# Autodesk Inventor assembly: ACTUADOR_LINEAL
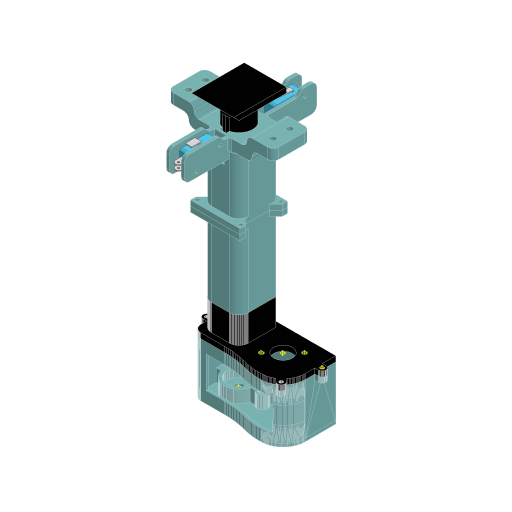
[picture p0: Inventor's stored thumbnail of the model, 512x512]
Saved by Autodesk Inventor 2024 (Build 280153000, 153)
## iProperties
Created: 2024-08-20
Part Number: ACTUADOR_LINEAL
Document SubType Name: Assembly
Designer: Jhuliams
Author: Jhuliams
## Documents named in this file (8)
- C:\Users\Jhuliams\Documents\GitHub\RECICLADOR_MODELO_3D\ACTUADOR_PARA_EMPUJAR_HACIA_ABAJO\ACTUADOR_LINEAL.iam
- C:\Users\Jhuliams\Documents\GitHub\RECICLADOR_MODELO_3D\ACTUADOR_PARA_EMPUJAR_HACIA_ABAJO\PART_1.ipt
- C:\Users\Jhuliams\Documents\GitHub\RECICLADOR_MODELO_3D\ACTUADOR_PARA_EMPUJAR_HACIA_ABAJO\PART_2.ipt
- C:\Users\Jhuliams\Documents\GitHub\RECICLADOR_MODELO_3D\ACTUADOR_PARA_EMPUJAR_HACIA_ABAJO\PART_4.ipt
- C:\Users\Jhuliams\Documents\GitHub\RECICLADOR_MODELO_3D\ACTUADOR_PARA_EMPUJAR_HACIA_ABAJO\PART_6.ipt
- C:\Users\Jhuliams\Documents\GitHub\RECICLADOR_MODELO_3D\ACTUADOR_PARA_EMPUJAR_HACIA_ABAJO\PART_5_1.ipt
- C:\Users\Jhuliams\Documents\GitHub\RECICLADOR_MODELO_3D\ACTUADOR_PARA_EMPUJAR_HACIA_ABAJO\CARCASA_NUEVA.ipt
- C:\Users\Jhuliams\Documents\GitHub\RECICLADOR_MODELO_3D\ACTUADOR_PARA_EMPUJAR_HACIA_ABAJO\FIN_DE_CARRERA.ipt
## Components (8 placed, 7 different names)
1. PART_1:1 — Flush:1, Flush:2, Mate:11, Mate:12
2. PART_2:1 — Flush:1, Flush:2, Mate:6, Flush:5, Mate:12, Flush:6, Flush:7, Flush:8, Mate:13
3. PART_4:1 — Mate:3, Mate:4, Mate:5, Flush:5
4. PART_6:1 — Mate:3, Mate:4, Mate:5, Mate:6, Mate:11
5. CARCASA_NUEVA:1 — Flush:6, Flush:7, Flush:8, Mate:13, Mate:18, Mate:19, Mate:20, Mate:21, Mate:22, Mate:23, Mate:24, Mate:25, Mate:26
6. PART_5_1:1 — Mate:18, Mate:19, Mate:20
7. FIN_DE_CARRERA:2 — Mate:21, Mate:22, Mate:23
8. FIN_DE_CARRERA:3 — Mate:24, Mate:25, Mate:26
## Relationships (22: Mate 16, Flush 6)
- Flush:1: PART_1:1 ↔ PART_2:1
- Flush:2: PART_1:1 ↔ PART_2:1
- Mate:3: PART_4:1 ↔ PART_6:1
- Mate:4: PART_4:1 ↔ PART_6:1
- Mate:5: PART_4:1 ↔ PART_6:1
- Mate:6: PART_2:1 ↔ PART_6:1
- Flush:5 (5 mm): PART_2:1 ↔ PART_4:1
- Mate:11: PART_1:1 ↔ PART_6:1
- Mate:12: PART_1:1 ↔ PART_2:1
- Flush:6: PART_2:1 ↔ CARCASA_NUEVA:1
- Flush:7: PART_2:1 ↔ CARCASA_NUEVA:1
- Flush:8: PART_2:1 ↔ CARCASA_NUEVA:1
- Mate:13: PART_2:1 ↔ CARCASA_NUEVA:1
- Mate:18 (0.25 mm): CARCASA_NUEVA:1 ↔ PART_5_1:1
- Mate:19 (0.25 mm): CARCASA_NUEVA:1 ↔ PART_5_1:1
- Mate:20 (0.75 mm): CARCASA_NUEVA:1 ↔ PART_5_1:1
- Mate:21: CARCASA_NUEVA:1 ↔ FIN_DE_CARRERA:2
- Mate:22: CARCASA_NUEVA:1 ↔ FIN_DE_CARRERA:2
- Mate:23 (0.5 mm): CARCASA_NUEVA:1 ↔ FIN_DE_CARRERA:2
- Mate:24: CARCASA_NUEVA:1 ↔ FIN_DE_CARRERA:3
- Mate:25: CARCASA_NUEVA:1 ↔ FIN_DE_CARRERA:3
- Mate:26 (0.5 mm): CARCASA_NUEVA:1 ↔ FIN_DE_CARRERA:3
